# Autodesk Inventor assembly: FullApparatus
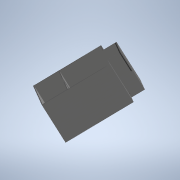
[picture p0: Inventor's stored thumbnail of the model, 180x180]
Saved by Autodesk Inventor 2020 (Build 240168000, 168)
## iProperties
Created: 2019-09-17
Part Number: FullApparatus
Document SubType Name: Assembly
Designer: Knowblesse
Author: Knowblesse
## Documents named in this file (4)
- C:\VCF\Lobster\Apparatus\Visual\FullApparatus.iam
- C:\VCF\Lobster\Apparatus\Visual\Main.ipt
- C:\VCF\Lobster\Apparatus\Visual\Motor_Panel.iam
- C:\VCF\Lobster\Apparatus\Visual\IRLight.ipt
## Components (3 placed, 3 different names)
1. Main:1 — 강체:1, 강체:2
2. Motor_Panel:1 [sub-assembly] — 강체:1
3. IRLight:1 — 강체:2
## Relationships (2: WeldJoint 2)
- 강체:1 [WeldJoint]: Main:1 ↔ Motor_Panel:1
- 강체:2 [WeldJoint]: Main:1 ↔ IRLight:1
